# Autodesk Inventor assembly: inner_MIR
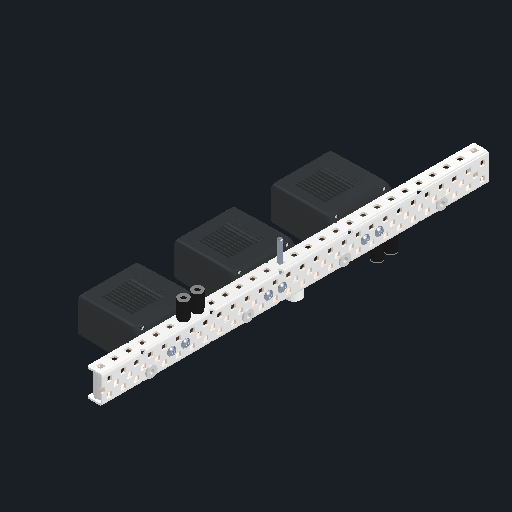
[picture p0: Inventor's stored thumbnail of the model, 512x512]
Saved by Autodesk Inventor 2024 (Build 280153000, 153)
## iProperties
Created: 2023-10-29
Part Number: inner_MIR
Document SubType Name: Assembly
Designer: avere
Author: avere
## Documents named in this file (15)
- C:\Users\avere\Documents\rbp_cad\zoomba_v0.1\chassis\mirrored_parts\inner_MIR.iam
- C:\Users\avere\Documents\rbp_cad\zoomba_v0.1\chassis\mirrored_parts\Insert Circle_MIR.ipt
- C:\Users\avere\Documents\rbp_cad\zoomba_v0.1\chassis\mirrored_parts\Alu C 1x2x1x28_MIR.ipt
- C:\Users\avere\Documents\rbp_cad\zoomba_v0.1\chassis\mirrored_parts\SteelM-StarS_MIR.iam
- C:\Users\avere\Documents\rbp_cad\zoomba_v0.1\chassis\mirrored_parts\.375 OD Aluminum Spacer 0.875_MIR.ipt
- C:\Users\avere\Documents\rbp_cad\VEX-CAD-Inventor-1.41\Motion\Spacers\Spacer Nylon .375 OD.ipt
- C:\Users\avere\Documents\rbp_cad\zoomba_v0.1\chassis\drivebay\custom_parts\washer_thick.ipt
- C:\Users\avere\Documents\rbp_cad\VEX-CAD-Inventor-1.41\Motion\Spacers\Spacer Nylon .500 OD\NSpacer White .500 OD x .250.ipt
- C:\Users\avere\Documents\rbp_cad\VEX-CAD-Inventor-1.41\Motion\Spacers\Spacer Nylon .500 OD.ipt
- C:\Users\avere\Documents\rbp_cad\hardware\.375 OD Aluminum Spacer 0.875.ipt
- C:\Users\avere\Documents\rbp_cad\VEX-CAD-Inventor-1.41\Motion\Spacers\Spacer Nylon .375 OD\NSpacer .375 OD x .125.ipt
- C:\Users\avere\Documents\rbp_cad\VEX-CAD-Inventor-1.41\Motion\Spacers\Washer Steel.ipt
- C:\Users\avere\Documents\rbp_cad\VEX-CAD-Inventor-1.41\Motion\Spacers\Spacer Nylon .375 OD\NSpacer .375 OD x .500.ipt
- C:\Users\avere\Documents\rbp_cad\VEX-CAD-Inventor-1.41\Motion\Spacers\Washer Steel\SWasher .375 OD x .031250.ipt
- C:\Users\avere\Documents\rbp_cad\VEX-CAD-Inventor-1.41\Structure\Hardware\Screw Shoulder Robosource\SScrew Shoulder Smooth 1.750 x .04.ipt
## Components (25 placed, 11 different names)
1. Insert Circle_MIR:1 — Insert:1
2. Insert Circle_MIR:2 — Insert:2
3. Insert Circle_MIR:3 — Insert:3
4. Insert Circle_MIR:4 — Insert:4
5. Alu C 1x2x1x28_MIR:1 — Insert:2, Insert:1, Insert:4, Insert:3, Mate:1, Insert:5, Mate:2, Insert:6, Mate:3, Insert:7, Insert:8, Insert:18, Insert:19, Insert:33, Insert:34, Insert:35, Insert:40, Insert:41
6. SteelM-StarS_MIR:1 [sub-assembly] — Mate:1, Insert:5
7. SteelM-StarS_MIR:2 [sub-assembly] — Mate:2, Insert:6
8. SteelM-StarS_MIR:3 [sub-assembly] — Mate:3, Insert:7
9. .375 OD Aluminum Spacer 0.875_MIR:1 — Insert:8
10. washer_thick:1 — Insert:18
11. NSpacer White .500 OD x .250:1
12. .375 OD Aluminum Spacer 0.875:1 — Insert:19
13. NSpacer .375 OD x .500:6 — Insert:33
14. NSpacer .375 OD x .125:7
15. SWasher .375 OD x .031250:5
16. NSpacer .375 OD x .500:8 — Insert:34
17. NSpacer .375 OD x .125:9
18. SWasher .375 OD x .031250:6
19. SScrew Shoulder Smooth 1.750 x .04:1 — Insert:35
20. NSpacer .375 OD x .500:10 — Insert:40
21. NSpacer .375 OD x .125:11
22. SWasher .375 OD x .031250:7
23. NSpacer .375 OD x .500:12 — Insert:41
24. NSpacer .375 OD x .125:13
25. SWasher .375 OD x .031250:8
## Relationships (27: Insert 24, Mate 3)
- Insert:2: Insert Circle_MIR:2 ↔ Alu C 1x2x1x28_MIR:1
- Insert:1: Insert Circle_MIR:1 ↔ Alu C 1x2x1x28_MIR:1
- Insert:4: Insert Circle_MIR:4 ↔ Alu C 1x2x1x28_MIR:1
- Insert:3: Insert Circle_MIR:3 ↔ Alu C 1x2x1x28_MIR:1
- Mate:1: Alu C 1x2x1x28_MIR:1 ↔ SteelM-StarS_MIR:1
- Insert:5: Alu C 1x2x1x28_MIR:1 ↔ SteelM-StarS_MIR:1
- Mate:2: Alu C 1x2x1x28_MIR:1 ↔ SteelM-StarS_MIR:2
- Insert:6: Alu C 1x2x1x28_MIR:1 ↔ SteelM-StarS_MIR:2
- Mate:3: Alu C 1x2x1x28_MIR:1 ↔ SteelM-StarS_MIR:3
- Insert:7: Alu C 1x2x1x28_MIR:1 ↔ SteelM-StarS_MIR:3
- Insert:8: Alu C 1x2x1x28_MIR:1 ↔ .375 OD Aluminum Spacer 0.875_MIR:1
- [Insert]: washer_thick:1 ↔ NSpacer White .500 OD x .250:1
- Insert:18: Alu C 1x2x1x28_MIR:1 ↔ washer_thick:1
- Insert:19: Alu C 1x2x1x28_MIR:1 ↔ .375 OD Aluminum Spacer 0.875:1
- [Insert]: NSpacer .375 OD x .500:6 ↔ NSpacer .375 OD x .125:7
- [Insert]: NSpacer .375 OD x .125:7 ↔ SWasher .375 OD x .031250:5
- [Insert]: NSpacer .375 OD x .500:8 ↔ NSpacer .375 OD x .125:9
- [Insert]: NSpacer .375 OD x .125:9 ↔ SWasher .375 OD x .031250:6
- Insert:33: Alu C 1x2x1x28_MIR:1 ↔ NSpacer .375 OD x .500:6
- Insert:34: Alu C 1x2x1x28_MIR:1 ↔ NSpacer .375 OD x .500:8
- Insert:35: Alu C 1x2x1x28_MIR:1 ↔ SScrew Shoulder Smooth 1.750 x .04:1
- [Insert]: NSpacer .375 OD x .500:10 ↔ NSpacer .375 OD x .125:11
- [Insert]: NSpacer .375 OD x .125:11 ↔ SWasher .375 OD x .031250:7
- [Insert]: NSpacer .375 OD x .500:12 ↔ NSpacer .375 OD x .125:13
- [Insert]: NSpacer .375 OD x .125:13 ↔ SWasher .375 OD x .031250:8
- Insert:40: Alu C 1x2x1x28_MIR:1 ↔ NSpacer .375 OD x .500:10
- Insert:41: Alu C 1x2x1x28_MIR:1 ↔ NSpacer .375 OD x .500:12
## Named parameters: d31_d25 = 0 mm, d32_d26 = 0 mm, d33_d25 = 0 mm, d34_d26 = 0 mm, d38_d27_d25 = 0 mm, d39_d28_d26 = 0 mm, d40_d27_d25 = 0 mm, d41_d28_d26 = 0 mm
